# Autodesk Inventor assembly: llanta trasera
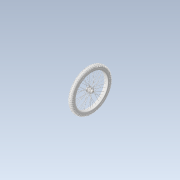
[picture p0: Inventor's stored thumbnail of the model, 180x180]
Saved by Autodesk Inventor 2021 (Build 250183000, 183)
## iProperties
Created: 2021-04-24
Part Number: llanta trasera
Document SubType Name: Assembly
Designer: j2seb
Author: j2seb
## Documents named in this file (3)
- G:\Unidades compartidas\APM\02 Inventor-Drive\llanta trasera.iam
- G:\Unidades compartidas\APM\02 Inventor-Drive\Ensamble_Llanta.iam
- G:\Unidades compartidas\APM\02 Inventor-Drive\eje manzana.ipt
## Components (2 placed, 2 different names)
1. Ensamble_Llanta:1 [sub-assembly] — Coincidencia:1
2. eje manzana:1 — Coincidencia:1
## Relationships (1: Mate 1)
- Coincidencia:1 [Mate]: Ensamble_Llanta:1 ↔ eje manzana:1
